# Autodesk Inventor assembly: Final Assembly
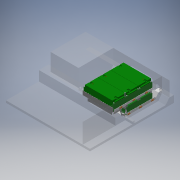
[picture p0: Inventor's stored thumbnail of the model, 180x180]
Saved by Autodesk Inventor 2017 (Build 210142000, 142)
## iProperties
Created: 2022-08-16
Part Number: Final Assembly
Document SubType Name: Assembly
Designer: JTS
Author: JTS
## Documents named in this file (22)
- C:\Users\Win240\Desktop\47 Ah FoMoCo Tray\RevB\02 Final Assembly (Tray Mated).iam
- C:\Users\Win240\Desktop\47 Ah FoMoCo Tray\RevB\LiBCM003 - Battery Tray\47 Ah FoMoCo Aluminum Tray.ipt
- C:\Users\Win240\Desktop\47 Ah FoMoCo Tray\RevB\OEM Parts\Junction Board.ipt
- C:\Users\Win240\Desktop\47 Ah FoMoCo Tray\RevB\OEM Parts\MCM.ipt
- C:\Users\Win240\Desktop\47 Ah FoMoCo Tray\RevB\Battery Modules\47Ah-FoMoCo.ipt
- C:\Users\Win240\Desktop\47 Ah FoMoCo Tray\RevB\LiBCM004 - Battery Rail\Bracket - 5th Module 8982K875.ipt
- C:\Users\Win240\Desktop\47 Ah FoMoCo Tray\RevB\LiBCM PCB\LiBCM Safety Cover - RevC.ipt
- C:\Users\Win240\Desktop\47 Ah FoMoCo Tray\RevB\LiBCM PCB\PCB.ipt
- C:\Users\Win240\Desktop\47 Ah FoMoCo Tray\RevB\OEM Parts\IMA Bay - Battery Enclosure Interface.ipt
- C:\Users\Win240\Desktop\47 Ah FoMoCo Tray\RevB\Nuts & Bolts\Battery Bolt.iam
- C:\Users\Win240\Desktop\47 Ah FoMoCo Tray\RevB\Nuts & Bolts\Threaded Standoff.ipt
- C:\Users\Win240\Desktop\47 Ah FoMoCo Tray\RevB\Nuts & Bolts\Battery Bolt - Split Washer.iam
- C:\Users\Win240\Desktop\47 Ah FoMoCo Tray\RevB\Nuts & Bolts\Washer 0.250in 92141A029.ipt
- C:\Users\Win240\Desktop\47 Ah FoMoCo Tray\RevB\Nuts & Bolts\Nut - Hex - 0.250in-20 91845A029.ipt
- C:\Users\Win240\Desktop\47 Ah FoMoCo Tray\RevB\Nuts & Bolts\Top Spacer.ipt
- C:\Users\Win240\Desktop\47 Ah FoMoCo Tray\RevB\Nuts & Bolts\PEMSERT.ipt
- C:\Users\Win240\Desktop\47 Ah FoMoCo Tray\RevB\Grid Chargers\UHP-1500-230.ipt
- C:\Users\Win240\Desktop\47 Ah FoMoCo Tray\RevB\Grid Chargers\HLG-480H-C2100B.ipt
- C:\Users\Win240\Desktop\47 Ah FoMoCo Tray\RevB\LiBCM005 - Charger Mount\Charger Mount.ipt
- C:\Users\Win240\Desktop\47 Ah FoMoCo Tray\RevB\Grid Chargers\HLG-240H-C1050B.ipt
- C:\Users\Win240\Desktop\47 Ah FoMoCo Tray\RevB\Nuts & Bolts\Fan.ipt
- C:\Users\Win240\Desktop\47 Ah FoMoCo Tray\RevB\Nuts & Bolts\Power Resistor - HSA25.ipt
## Components (73 placed, 21 different names)
1. IMA Bay - Battery Enclosure Interface:1 — Insert:56, Mate:2, Mate:3, Mate:4
2. Junction Board:1 — Insert:11, Insert:12
3. MCM:1 — Insert:137, Insert:138
4. Washer 0.250in 92141A029:3 — Insert:124
5. Nut - Hex - 0.250in-20 91845A029:5
6. Top Spacer:1 — Insert:125, Insert:126
7. PEMSERT:1 — Insert:129
8. PEMSERT:2 — Insert:130
9. PEMSERT:3 — Insert:131
10. PEMSERT:4 — Insert:132
11. UHP-1500-230:1 — Mate:5, Mate:6, Flush:2, Flush:8, Flush:9
12. HLG-240H-C1050B:1 — Mate:8, Flush:10, Flush:11
13. HLG-480H-C2100B:1 — Mate:7, Flush:8, Flush:9, Flush:10, Flush:11
14. Charger Mount:1 — Flush:5, Flush:6, Mate:8, Insert:133, Insert:134
15. Fan:1 — Insert:133, Insert:134
16. Top Spacer:2 — Insert:135, Insert:138
17. Top Spacer:3 — Insert:136, Insert:137
18. 47 Ah FoMoCo Aluminum Tray:1 — Insert:11, Insert:12, Insert:56, Mate:2, Insert:97, Insert:98, Insert:99, Insert:100, Insert:101, Insert:102, Insert:103, Insert:104, Insert:105, Insert:106, Insert:107, Insert:108, Insert:124, Insert:135, Insert:136, Insert:151, Insert:152, Insert:153, Insert:154, Insert:155, Insert:156, Insert:157, Insert:158, Insert:159, Insert:160, Insert:161, Insert:162, Insert:163, Insert:164, Insert:165, Insert:166, Insert:167, Insert:168, Insert:169, Insert:170, Insert:171, Insert:172, Insert:173, Insert:174
19. LiBCM Safety Cover - RevC:1 — Insert:55, Mate:1, Mate:3, Flush:1, Mate:4
20. PCB:1 — Insert:55, Mate:1
21. Threaded Standoff:1 — Insert:65
22. Threaded Standoff:2 — Insert:70
23. Threaded Standoff:3 — Insert:71
24. Threaded Standoff:4 — Insert:72, Insert:114
25. Threaded Standoff:5 — Insert:69, Insert:113
26. Threaded Standoff:6 — Insert:68, Insert:110
27. Threaded Standoff:7 — Insert:67
28. Threaded Standoff:8 — Insert:66, Insert:109
29. Battery Bolt:1 [sub-assembly] — Insert:102
30. Battery Bolt:2 [sub-assembly] — Insert:101
31. Battery Bolt:3 [sub-assembly] — Insert:99
32. Battery Bolt:4 [sub-assembly] — Insert:98
33. Battery Bolt:5 [sub-assembly] — Insert:100
34. Battery Bolt:6 [sub-assembly] — Insert:104
35. Battery Bolt:7 [sub-assembly] — Insert:103
36. Battery Bolt:8 [sub-assembly] — Insert:97
37. 47Ah-FoMoCo:1 — Insert:65, Insert:66, Insert:71, Insert:72, Insert:107, Insert:108
38. 47Ah-FoMoCo:2 — Insert:67, Insert:68, Insert:69, Insert:70, Insert:105, Insert:106
39. Bracket - 5th Module 8982K875:1 — Insert:109, Insert:110, Insert:120, Insert:121, Insert:122, Insert:131, Insert:132, Mate:5, Mate:6, Flush:2, Mate:7, Insert:145, Insert:146, Insert:147, Insert:148, Insert:149, Insert:150
40. Bracket - 5th Module 8982K875:2 — Insert:113, Insert:114, Insert:117, Insert:118, Insert:119, Insert:129, Insert:130, Flush:5, Flush:6, Insert:139, Insert:140, Insert:141, Insert:142, Insert:143, Insert:144
41. Battery Bolt:9 [sub-assembly] — Insert:127
42. Battery Bolt:10 [sub-assembly] — Insert:128
43. Battery Bolt - Split Washer:1 [sub-assembly] — Insert:77
44. Battery Bolt - Split Washer:2 [sub-assembly] — Insert:78
45. Battery Bolt - Split Washer:3 [sub-assembly] — Insert:79
46. Battery Bolt - Split Washer:4 [sub-assembly] — Insert:80
47. Battery Bolt - Split Washer:5 [sub-assembly] — Insert:84
48. Battery Bolt - Split Washer:6 [sub-assembly] — Insert:83
49. Battery Bolt - Split Washer:7 [sub-assembly] — Insert:82
50. Battery Bolt - Split Washer:8 [sub-assembly] — Insert:81
51. Battery Bolt - Split Washer:9 [sub-assembly] — Insert:126
52. Battery Bolt - Split Washer:10 [sub-assembly] — Insert:85
53. 47Ah-FoMoCo:3 — Flush:1, Insert:79, Insert:80, Insert:81, Insert:82, Insert:121, Insert:122
54. 47Ah-FoMoCo:4 — Insert:77, Insert:78, Insert:83, Insert:84, Insert:119, Insert:120
55. 47Ah-FoMoCo:5 — Insert:85, Insert:117, Insert:118, Insert:125, Insert:127, Insert:128
56. Power Resistor - HSA25:20 — Insert:159, Insert:160
57. Power Resistor - HSA25:10 — Insert:157, Insert:158
58. Power Resistor - HSA25:16 — Insert:163, Insert:164
59. Power Resistor - HSA25:18 — Insert:167, Insert:168
60. Power Resistor - HSA25:15 — Insert:165, Insert:166
61. Power Resistor - HSA25:11 — Insert:161, Insert:162
62. Power Resistor - HSA25:9 — Insert:153, Insert:154
63. Power Resistor - HSA25:5 — Insert:173, Insert:174
64. Power Resistor - HSA25:6 — Insert:171, Insert:172
65. Power Resistor - HSA25:19 — Insert:151, Insert:152
66. Power Resistor - HSA25:4 — Insert:169, Insert:170
67. Power Resistor - HSA25:8 — Insert:155, Insert:156
68. Power Resistor - HSA25:3 — Insert:139, Insert:140
69. Power Resistor - HSA25:12 — Insert:147, Insert:148
70. Power Resistor - HSA25:13 — Insert:145, Insert:146
71. Power Resistor - HSA25:2 — Insert:141, Insert:142
72. Power Resistor - HSA25:1 — Insert:143, Insert:144
73. Power Resistor - HSA25:14 — Insert:149, Insert:150
## Relationships (111: Insert 95, Mate 8, Flush 8)
- Insert:11: Junction Board:1 ↔ 47 Ah FoMoCo Aluminum Tray:1
- Insert:12: Junction Board:1 ↔ 47 Ah FoMoCo Aluminum Tray:1
- Insert:55 (37 mm): LiBCM Safety Cover - RevC:1 ↔ PCB:1
- Mate:1: LiBCM Safety Cover - RevC:1 ↔ PCB:1
- Insert:56: IMA Bay - Battery Enclosure Interface:1 ↔ 47 Ah FoMoCo Aluminum Tray:1
- Mate:2: IMA Bay - Battery Enclosure Interface:1 ↔ 47 Ah FoMoCo Aluminum Tray:1
- Mate:3 (5 mm): IMA Bay - Battery Enclosure Interface:1 ↔ LiBCM Safety Cover - RevC:1
- Flush:1 (45 mm): LiBCM Safety Cover - RevC:1 ↔ 47Ah-FoMoCo:3
- Mate:4 (31.5 mm): IMA Bay - Battery Enclosure Interface:1 ↔ LiBCM Safety Cover - RevC:1
- Insert:65: Threaded Standoff:1 ↔ 47Ah-FoMoCo:1
- Insert:66: Threaded Standoff:8 ↔ 47Ah-FoMoCo:1
- Insert:67: Threaded Standoff:7 ↔ 47Ah-FoMoCo:2
- Insert:68: Threaded Standoff:6 ↔ 47Ah-FoMoCo:2
- Insert:69: Threaded Standoff:5 ↔ 47Ah-FoMoCo:2
- Insert:70: Threaded Standoff:2 ↔ 47Ah-FoMoCo:2
- Insert:71: Threaded Standoff:3 ↔ 47Ah-FoMoCo:1
- Insert:72: Threaded Standoff:4 ↔ 47Ah-FoMoCo:1
- Insert:77: Battery Bolt - Split Washer:1 ↔ 47Ah-FoMoCo:4
- Insert:78: Battery Bolt - Split Washer:2 ↔ 47Ah-FoMoCo:4
- Insert:79: Battery Bolt - Split Washer:3 ↔ 47Ah-FoMoCo:3
- Insert:80: Battery Bolt - Split Washer:4 ↔ 47Ah-FoMoCo:3
- Insert:81: Battery Bolt - Split Washer:8 ↔ 47Ah-FoMoCo:3
- Insert:82: Battery Bolt - Split Washer:7 ↔ 47Ah-FoMoCo:3
- Insert:83: Battery Bolt - Split Washer:6 ↔ 47Ah-FoMoCo:4
- Insert:84: Battery Bolt - Split Washer:5 ↔ 47Ah-FoMoCo:4
- Insert:85: Battery Bolt - Split Washer:10 ↔ 47Ah-FoMoCo:5
- Insert:97: 47 Ah FoMoCo Aluminum Tray:1 ↔ Battery Bolt:8
- Insert:98: 47 Ah FoMoCo Aluminum Tray:1 ↔ Battery Bolt:4
- Insert:99: 47 Ah FoMoCo Aluminum Tray:1 ↔ Battery Bolt:3
- Insert:100: 47 Ah FoMoCo Aluminum Tray:1 ↔ Battery Bolt:5
- Insert:101: 47 Ah FoMoCo Aluminum Tray:1 ↔ Battery Bolt:2
- Insert:102: 47 Ah FoMoCo Aluminum Tray:1 ↔ Battery Bolt:1
- Insert:103: 47 Ah FoMoCo Aluminum Tray:1 ↔ Battery Bolt:7
- Insert:104: 47 Ah FoMoCo Aluminum Tray:1 ↔ Battery Bolt:6
- Insert:105: 47 Ah FoMoCo Aluminum Tray:1 ↔ 47Ah-FoMoCo:2
- Insert:106: 47 Ah FoMoCo Aluminum Tray:1 ↔ 47Ah-FoMoCo:2
- Insert:107: 47 Ah FoMoCo Aluminum Tray:1 ↔ 47Ah-FoMoCo:1
- Insert:108: 47 Ah FoMoCo Aluminum Tray:1 ↔ 47Ah-FoMoCo:1
- Insert:109: Threaded Standoff:8 ↔ Bracket - 5th Module 8982K875:1
- Insert:110: Threaded Standoff:6 ↔ Bracket - 5th Module 8982K875:1
- Insert:113: Threaded Standoff:5 ↔ Bracket - 5th Module 8982K875:2
- Insert:114: Threaded Standoff:4 ↔ Bracket - 5th Module 8982K875:2
- Insert:117: Bracket - 5th Module 8982K875:2 ↔ 47Ah-FoMoCo:5
- Insert:118: Bracket - 5th Module 8982K875:2 ↔ 47Ah-FoMoCo:5
- Insert:119: Bracket - 5th Module 8982K875:2 ↔ 47Ah-FoMoCo:4
- Insert:120: Bracket - 5th Module 8982K875:1 ↔ 47Ah-FoMoCo:4
- Insert:121: Bracket - 5th Module 8982K875:1 ↔ 47Ah-FoMoCo:3
- Insert:122: Bracket - 5th Module 8982K875:1 ↔ 47Ah-FoMoCo:3
- [Insert]: Washer 0.250in 92141A029:3 ↔ Nut - Hex - 0.250in-20 91845A029:5
- Insert:124: Washer 0.250in 92141A029:3 ↔ 47 Ah FoMoCo Aluminum Tray:1
- Insert:125: Top Spacer:1 ↔ 47Ah-FoMoCo:5
- Insert:126: Top Spacer:1 ↔ Battery Bolt - Split Washer:9
- Insert:127: Battery Bolt:9 ↔ 47Ah-FoMoCo:5
- Insert:128: Battery Bolt:10 ↔ 47Ah-FoMoCo:5
- Insert:129: PEMSERT:1 ↔ Bracket - 5th Module 8982K875:2
- Insert:130: PEMSERT:2 ↔ Bracket - 5th Module 8982K875:2
- Insert:131: PEMSERT:3 ↔ Bracket - 5th Module 8982K875:1
- Insert:132: PEMSERT:4 ↔ Bracket - 5th Module 8982K875:1
- Mate:5: UHP-1500-230:1 ↔ Bracket - 5th Module 8982K875:1
- Mate:6 (1 mm): UHP-1500-230:1 ↔ Bracket - 5th Module 8982K875:1
- Flush:2: UHP-1500-230:1 ↔ Bracket - 5th Module 8982K875:1
- Mate:7: HLG-480H-C2100B:1 ↔ Bracket - 5th Module 8982K875:1
- Flush:5: Charger Mount:1 ↔ Bracket - 5th Module 8982K875:2
- Flush:6: Charger Mount:1 ↔ Bracket - 5th Module 8982K875:2
- Mate:8: HLG-240H-C1050B:1 ↔ Charger Mount:1
- Flush:8: UHP-1500-230:1 ↔ HLG-480H-C2100B:1
- Flush:9: UHP-1500-230:1 ↔ HLG-480H-C2100B:1
- Flush:10: HLG-240H-C1050B:1 ↔ HLG-480H-C2100B:1
- Flush:11: HLG-240H-C1050B:1 ↔ HLG-480H-C2100B:1
- Insert:133: Charger Mount:1 ↔ Fan:1
- Insert:134: Charger Mount:1 ↔ Fan:1
- Insert:135: Top Spacer:2 ↔ 47 Ah FoMoCo Aluminum Tray:1
- Insert:136: Top Spacer:3 ↔ 47 Ah FoMoCo Aluminum Tray:1
- Insert:137: MCM:1 ↔ Top Spacer:3
- Insert:138: MCM:1 ↔ Top Spacer:2
- Insert:139: Bracket - 5th Module 8982K875:2 ↔ Power Resistor - HSA25:3
- Insert:140: Bracket - 5th Module 8982K875:2 ↔ Power Resistor - HSA25:3
- Insert:141: Bracket - 5th Module 8982K875:2 ↔ Power Resistor - HSA25:2
- Insert:142: Bracket - 5th Module 8982K875:2 ↔ Power Resistor - HSA25:2
- Insert:143: Bracket - 5th Module 8982K875:2 ↔ Power Resistor - HSA25:1
- Insert:144: Bracket - 5th Module 8982K875:2 ↔ Power Resistor - HSA25:1
- Insert:145: Bracket - 5th Module 8982K875:1 ↔ Power Resistor - HSA25:13
- Insert:146: Bracket - 5th Module 8982K875:1 ↔ Power Resistor - HSA25:13
- Insert:147: Bracket - 5th Module 8982K875:1 ↔ Power Resistor - HSA25:12
- Insert:148: Bracket - 5th Module 8982K875:1 ↔ Power Resistor - HSA25:12
- Insert:149: Bracket - 5th Module 8982K875:1 ↔ Power Resistor - HSA25:14
- Insert:150: Bracket - 5th Module 8982K875:1 ↔ Power Resistor - HSA25:14
- Insert:151: 47 Ah FoMoCo Aluminum Tray:1 ↔ Power Resistor - HSA25:19
- Insert:152: 47 Ah FoMoCo Aluminum Tray:1 ↔ Power Resistor - HSA25:19
- Insert:153: 47 Ah FoMoCo Aluminum Tray:1 ↔ Power Resistor - HSA25:9
- Insert:154: 47 Ah FoMoCo Aluminum Tray:1 ↔ Power Resistor - HSA25:9
- Insert:155: 47 Ah FoMoCo Aluminum Tray:1 ↔ Power Resistor - HSA25:8
- Insert:156: 47 Ah FoMoCo Aluminum Tray:1 ↔ Power Resistor - HSA25:8
- Insert:157: 47 Ah FoMoCo Aluminum Tray:1 ↔ Power Resistor - HSA25:10
- Insert:158: 47 Ah FoMoCo Aluminum Tray:1 ↔ Power Resistor - HSA25:10
- Insert:159: 47 Ah FoMoCo Aluminum Tray:1 ↔ Power Resistor - HSA25:20
- Insert:160: 47 Ah FoMoCo Aluminum Tray:1 ↔ Power Resistor - HSA25:20
- Insert:161: 47 Ah FoMoCo Aluminum Tray:1 ↔ Power Resistor - HSA25:11
- Insert:162: 47 Ah FoMoCo Aluminum Tray:1 ↔ Power Resistor - HSA25:11
- Insert:163: 47 Ah FoMoCo Aluminum Tray:1 ↔ Power Resistor - HSA25:16
- Insert:164: 47 Ah FoMoCo Aluminum Tray:1 ↔ Power Resistor - HSA25:16
- Insert:165: 47 Ah FoMoCo Aluminum Tray:1 ↔ Power Resistor - HSA25:15
- Insert:166: 47 Ah FoMoCo Aluminum Tray:1 ↔ Power Resistor - HSA25:15
- Insert:167: 47 Ah FoMoCo Aluminum Tray:1 ↔ Power Resistor - HSA25:18
- Insert:168: 47 Ah FoMoCo Aluminum Tray:1 ↔ Power Resistor - HSA25:18
- Insert:169: 47 Ah FoMoCo Aluminum Tray:1 ↔ Power Resistor - HSA25:4
- Insert:170: 47 Ah FoMoCo Aluminum Tray:1 ↔ Power Resistor - HSA25:4
- Insert:171: 47 Ah FoMoCo Aluminum Tray:1 ↔ Power Resistor - HSA25:6
- Insert:172: 47 Ah FoMoCo Aluminum Tray:1 ↔ Power Resistor - HSA25:6
- Insert:173: 47 Ah FoMoCo Aluminum Tray:1 ↔ Power Resistor - HSA25:5
- Insert:174: 47 Ah FoMoCo Aluminum Tray:1 ↔ Power Resistor - HSA25:5
## Named parameters: d147_d115 = 0 mm
